# Autodesk Inventor assembly: COM_01
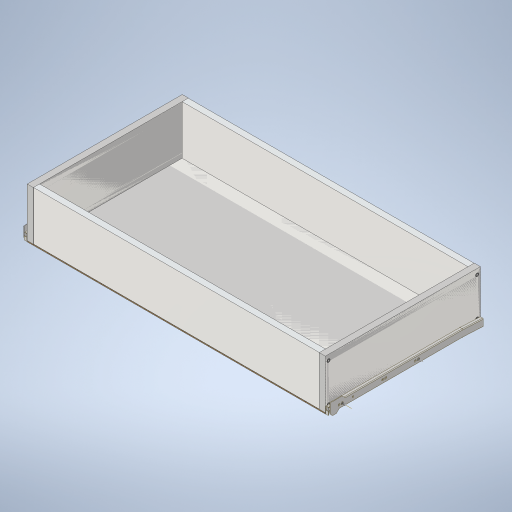
[picture p0: Inventor's stored thumbnail of the model, 512x512]
Saved by Autodesk Inventor 2024 (Build 280153000, 153)
## iProperties
RuleStatus: InUse
Created: 2015-02-10
Part Number: COM_01
Document SubType Name: Assembly
Designer: SauliusD
Description: Partial Pull Drawer 30 kg
AfterAnyParamChange0: Screw Positioning and Ammount Control
AfterAnyParamChange1: Change Skeleton Parameters
Author: SauliusD
## Documents named in this file (15)
- C:\W4INV 2024 Design\PROJECTS\Samples\Commode\CommodePartial Pull Drawer 30 kg1\COM_01.iam
- C:\W4INV 2024 Design\PROJECTS\Samples\Commode\CommodePartial Pull Drawer 30 kg1\COM_0104.ipt
- C:\W4INV 2024 Design\PROJECTS\Samples\Commode\CommodePartial Pull Drawer 30 kg1\COM_0106.ipt
- C:\W4INV 2024 Design\PROJECTS\Samples\Commode\CommodePartial Pull Drawer 30 kg1\COM_0107.ipt
- C:\W4INV 2024 Design\PROJECTS\Samples\Commode\CommodePartial Pull Drawer 30 kg1\COM_0102.ipt
- C:\W4INV 2024 Design\PROJECTS\Samples\Commode\CommodePartial Pull Drawer 30 kg1\COM_0103.ipt
- C:\W4INV 2024 Design\PROJECTS\Samples\Commode\CommodePartial Pull Drawer 30 kg1\COM_0110.ipt
- C:\W4INV 2024 Design\PROJECTS\Samples\Commode\CommodePartial Pull Drawer 30 kg1\COM_0109.ipt
- C:\W4INV 2024 Design\PROJECTS\Samples\Commode\CommodePartial Pull Drawer 30 kg1\COM_0105.ipt
- C:\W4INV 2024 Design\PROJECTS\Samples\Commode\CommodePartial Pull Drawer 30 kg1\COM_0108.ipt
- C:\W4INV 2024 Design\PROJECTS\Samples\Commode\CommodePartial Pull Drawer 30 kg1\SKL_COM_0101.ipt
- C:\W4INV 2024 Design\_LIBRARY\Fixed joints\Confirmat\CONFIRMAT\Confirmat L50 NB T18 PB T 18.ipt
- C:\W4INV 2024 Design\_LIBRARY\Fixed joints\Screws\WOOD SCREW CROSS RECESSED FLAT HEAD\Wood screw Cross Recessed Flat Head M3.5x16 H.ipt
- C:\W4INV 2022 Design\LIBRARY\Fixed joints\Screws\WOOD SCREW CROSS RECESSED FLAT HEAD.ipt
- C:\W4INV 2024 Design\LIBRARY\Fixed joints\Confirmat\CONFIRMAT.ipt
## Components (26 placed, 12 different names)
1. @Skeleton — Flush:1, Flush:2, Flush:3
2. COM_0104:1 — Axis Plane:1, Pillar Board Side Plane:1, Axis Plane:2, Pillar Board Side Plane:2, Axis Plane:3, Axis Plane:4, Axis Plane:5, Pillar Board Side Plane:5, Axis Plane:6, Pillar Board Side Plane:6, Axis Plane:7, Axis Plane:8
3. COM_0106:1 — Nestled Board Plane:1, Nestled Board Plane:3, Nestled Board Plane:5, Nestled Board Plane:7
4. COM_0107:1 — Nestled Board Plane:2, Nestled Board Plane:4, Nestled Board Plane:6, Nestled Board Plane:8
5. COM_0102:1 — Pillar Board Side Plane:3, Pillar Board Side Plane:4, Pillar Board Side Plane:7, Pillar Board Side Plane:8
6. COM_0103:1
7. COM_0110:1 — Insert:2, Insert:3
8. COM_0109:1 — Insert:1
9. COM_0105:1 — Insert:6
10. COM_0108:1 — Insert:4, Insert:5
11. Wood screw Cross Recessed Flat Head M3.5x16 H:9 — Insert:2
12. Wood screw Cross Recessed Flat Head M3.5x16 H:10 — Insert:3
13. Wood screw Cross Recessed Flat Head M3.5x16 H:11 — Insert:4
14. Wood screw Cross Recessed Flat Head M3.5x16 H:12 — Insert:5
15. Confirmat L50 NB T18 PB T 18:2 — Axis Plane:1, Pillar Board Side Plane:1, Nestled Board Plane:1
16. Confirmat L50 NB T18 PB T 18:3 — Axis Plane:2, Pillar Board Side Plane:2, Nestled Board Plane:2
17. Confirmat L50 NB T18 PB T 18:4 — Axis Plane:3, Pillar Board Side Plane:3, Nestled Board Plane:3
18. Confirmat L50 NB T18 PB T 18:5 — Axis Plane:4, Pillar Board Side Plane:4, Nestled Board Plane:4
19. Confirmat L50 NB T18 PB T 18:6 — Axis Plane:5, Pillar Board Side Plane:5, Nestled Board Plane:5
20. Confirmat L50 NB T18 PB T 18:7 — Axis Plane:6, Pillar Board Side Plane:6, Nestled Board Plane:6
21. Confirmat L50 NB T18 PB T 18:8 — Axis Plane:7, Pillar Board Side Plane:7, Nestled Board Plane:7
22. Confirmat L50 NB T18 PB T 18:9 — Axis Plane:8, Pillar Board Side Plane:8, Nestled Board Plane:8
23. Wood screw Cross Recessed Flat Head M3.5x16 H:13 — Insert:1
24. Wood screw Cross Recessed Flat Head M3.5x16 H:14
25. Wood screw Cross Recessed Flat Head M3.5x16 H:15 — Insert:6
26. Wood screw Cross Recessed Flat Head M3.5x16 H:16
## Component patterns: (2 elements, first: Wood screw Cross Recessed Flat Head M3.5x16 H:13), (2 elements, first: Wood screw Cross Recessed Flat Head M3.5x16 H:15)
## Relationships (33: Mate 16, Flush 11, Insert 6)
- Insert:1: COM_0109:1 ↔ Wood screw Cross Recessed Flat Head M3.5x16 H:13
- Flush:1: @Skeleton
- Flush:2: @Skeleton
- Flush:3: @Skeleton
- Insert:2: COM_0110:1 ↔ Wood screw Cross Recessed Flat Head M3.5x16 H:9
- Insert:3: COM_0110:1 ↔ Wood screw Cross Recessed Flat Head M3.5x16 H:10
- Insert:4: COM_0108:1 ↔ Wood screw Cross Recessed Flat Head M3.5x16 H:11
- Insert:5: COM_0108:1 ↔ Wood screw Cross Recessed Flat Head M3.5x16 H:12
- Insert:6: COM_0105:1 ↔ Wood screw Cross Recessed Flat Head M3.5x16 H:15
- Axis Plane:1 [Mate]: COM_0104:1 ↔ Confirmat L50 NB T18 PB T 18:2
- Pillar Board Side Plane:1 [Mate] (-9 mm): COM_0104:1 ↔ Confirmat L50 NB T18 PB T 18:2
- Nestled Board Plane:1 [Flush]: COM_0106:1 ↔ Confirmat L50 NB T18 PB T 18:2
- Axis Plane:2 [Mate]: COM_0104:1 ↔ Confirmat L50 NB T18 PB T 18:3
- Pillar Board Side Plane:2 [Mate] (-9 mm): COM_0104:1 ↔ Confirmat L50 NB T18 PB T 18:3
- Nestled Board Plane:2 [Flush]: COM_0107:1 ↔ Confirmat L50 NB T18 PB T 18:3
- Axis Plane:3 [Mate]: COM_0104:1 ↔ Confirmat L50 NB T18 PB T 18:4
- Pillar Board Side Plane:3 [Mate] (-9 mm): COM_0102:1 ↔ Confirmat L50 NB T18 PB T 18:4
- Nestled Board Plane:3 [Flush]: COM_0106:1 ↔ Confirmat L50 NB T18 PB T 18:4
- Axis Plane:4 [Mate]: COM_0104:1 ↔ Confirmat L50 NB T18 PB T 18:5
- Pillar Board Side Plane:4 [Mate] (-9 mm): COM_0102:1 ↔ Confirmat L50 NB T18 PB T 18:5
- Nestled Board Plane:4 [Flush]: COM_0107:1 ↔ Confirmat L50 NB T18 PB T 18:5
- Axis Plane:5 [Mate]: COM_0104:1 ↔ Confirmat L50 NB T18 PB T 18:6
- Pillar Board Side Plane:5 [Mate] (-9 mm): COM_0104:1 ↔ Confirmat L50 NB T18 PB T 18:6
- Nestled Board Plane:5 [Flush]: COM_0106:1 ↔ Confirmat L50 NB T18 PB T 18:6
- Axis Plane:6 [Mate]: COM_0104:1 ↔ Confirmat L50 NB T18 PB T 18:7
- Pillar Board Side Plane:6 [Mate] (-9 mm): COM_0104:1 ↔ Confirmat L50 NB T18 PB T 18:7
- Nestled Board Plane:6 [Flush]: COM_0107:1 ↔ Confirmat L50 NB T18 PB T 18:7
- Axis Plane:7 [Mate]: COM_0104:1 ↔ Confirmat L50 NB T18 PB T 18:8
- Pillar Board Side Plane:7 [Mate] (-9 mm): COM_0102:1 ↔ Confirmat L50 NB T18 PB T 18:8
- Nestled Board Plane:7 [Flush]: COM_0106:1 ↔ Confirmat L50 NB T18 PB T 18:8
- Axis Plane:8 [Mate]: COM_0104:1 ↔ Confirmat L50 NB T18 PB T 18:9
- Pillar Board Side Plane:8 [Mate] (-9 mm): COM_0102:1 ↔ Confirmat L50 NB T18 PB T 18:9
- Nestled Board Plane:8 [Flush]: COM_0107:1 ↔ Confirmat L50 NB T18 PB T 18:9
## Named parameters: Back_Screw_Position = 224 mm, iTrigger0 = 2, Drawer_H = 56 mm, Rear_Space = 20 mm, Facade_Inlet = 0.001 mm, Board_Thickness = 18 mm, Distance_from_bottom = 0 mm
